# Autodesk Inventor assembly: GE-12103
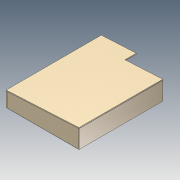
[picture p0: Inventor's stored thumbnail of the model, 180x180]
Saved by Autodesk Inventor 2012 (Build 160160000, 160)
## iProperties
Created: 2011-11-27
Part Number: GE-12103
Document SubType Name: Assembly
Designer: dfoster
Description: Fender, Assembly
Title: Fender, Assembly
Author: dfoster
## Documents named in this file (7)
- C:\Data Folder\FRC 2012 Field\Components\GE-12103.iam
- C:\Data Folder\FRC 2012 Field\Components\GE-12103-01.ipt
- C:\Data Folder\FRC 2012 Field\Components\GE-12103-02.ipt
- C:\Data Folder\FRC 2012 Field\Components\GE-12103-03.ipt
- C:\Data Folder\FRC 2012 Field\Components\GE-12103-04.ipt
- C:\Data Folder\FRC 2012 Field\Components\GE-12103-05.ipt
- C:\Data Folder\FRC 2012 Field\Components\GE-12103-06.ipt
## Components (13 placed, 6 different names)
1. GE-12103-01:1 — Mate:1, Flush:7, Flush:8, Flush:10, Flush:11, Flush:12, Mate:3, Mate:8, Mate:9, Mate:12, Mate:15, Flush:17, Flush:18
2. GE-12103-01:3 — Flush:1, Flush:6, Flush:10, Flush:11, Mate:9
3. GE-12103-01:4 — Flush:1, Flush:6, Flush:9, Flush:13, Mate:10, Mate:14, Mate:16
4. GE-12103-02:1 — Mate:1, Flush:7, Flush:8, Flush:9, Mate:2, Mate:5, Mate:6, Mate:7, Mate:11, Mate:17, Flush:20
5. GE-12103-03:1 — Mate:6, Mate:8, Flush:14, Flush:15
6. GE-12103-03:2 — Flush:13, Mate:5, Mate:14, Mate:18, Flush:19
7. GE-12103-03:3 — Flush:12, Mate:2, Mate:3, Mate:13, Flush:16, Mate:19, Flush:21
8. GE-12103-03:4 — Mate:7, Mate:10, Flush:14
9. GE-12103-03:5 — Mate:11, Mate:12, Mate:13, Flush:15
10. GE-12103-04:1 — Mate:15, Flush:16, Flush:17
11. GE-12103-05:1 — Mate:16, Flush:18, Mate:17
12. GE-12103-06:1 — Mate:18, Flush:19, Flush:20, Flush:22
13. GE-12103-06:2 — Mate:19, Flush:21, Flush:22
## Relationships (36: Flush 18, Mate 18)
- Flush:1: GE-12103-01:3 ↔ GE-12103-01:4
- Flush:6: GE-12103-01:3 ↔ GE-12103-01:4
- Mate:1: GE-12103-01:1 ↔ GE-12103-02:1
- Flush:7: GE-12103-01:1 ↔ GE-12103-02:1
- Flush:8: GE-12103-01:1 ↔ GE-12103-02:1
- Flush:9 (152.4 mm): GE-12103-01:4 ↔ GE-12103-02:1
- Flush:10: GE-12103-01:1 ↔ GE-12103-01:3
- Flush:11: GE-12103-01:1 ↔ GE-12103-01:3
- Flush:12: GE-12103-01:1 ↔ GE-12103-03:3
- Mate:2: GE-12103-02:1 ↔ GE-12103-03:3
- Mate:3: GE-12103-01:1 ↔ GE-12103-03:3
- Flush:13: GE-12103-01:4 ↔ GE-12103-03:2
- Mate:5: GE-12103-02:1 ↔ GE-12103-03:2
- Mate:6: GE-12103-02:1 ↔ GE-12103-03:1
- Mate:7: GE-12103-02:1 ↔ GE-12103-03:4
- Mate:8 (254 mm): GE-12103-01:1 ↔ GE-12103-03:1
- Mate:9 (542.925 mm): GE-12103-01:1 ↔ GE-12103-01:3
- Mate:10 (254 mm): GE-12103-01:4 ↔ GE-12103-03:4
- Flush:14: GE-12103-03:1 ↔ GE-12103-03:4
- Mate:11: GE-12103-02:1 ↔ GE-12103-03:5
- Mate:12: GE-12103-01:1 ↔ GE-12103-03:5
- Mate:13 (-190.5 mm): GE-12103-03:3 ↔ GE-12103-03:5
- Flush:15: GE-12103-03:1 ↔ GE-12103-03:5
- Mate:14: GE-12103-01:4 ↔ GE-12103-03:2
- Mate:15: GE-12103-01:1 ↔ GE-12103-04:1
- Flush:16: GE-12103-03:3 ↔ GE-12103-04:1
- Flush:17: GE-12103-01:1 ↔ GE-12103-04:1
- Mate:16: GE-12103-01:4 ↔ GE-12103-05:1
- Flush:18: GE-12103-01:1 ↔ GE-12103-05:1
- Mate:17: GE-12103-02:1 ↔ GE-12103-05:1
- Mate:18: GE-12103-03:2 ↔ GE-12103-06:1
- Flush:19: GE-12103-03:2 ↔ GE-12103-06:1
- Flush:20 (6.35 mm): GE-12103-02:1 ↔ GE-12103-06:1
- Mate:19: GE-12103-03:3 ↔ GE-12103-06:2
- Flush:21: GE-12103-03:3 ↔ GE-12103-06:2
- Flush:22: GE-12103-06:1 ↔ GE-12103-06:2
